# Autodesk Inventor assembly: Outer Wheel
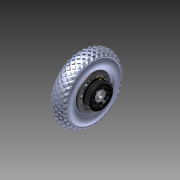
[picture p0: Inventor's stored thumbnail of the model, 180x180]
Saved by Autodesk Inventor 2014 SP1 (Build 180222100, 222)
## iProperties
Created: 2014-01-21
Part Number: Outer Wheel
Document SubType Name: Assembly
Designer: Nick
Author: Nick
## Documents named in this file (4)
- D:\Dropbox\School\PurdueFIRST\PFP Robot\PFP Robot with Cart\Outer Wheel.iam
- D:\Dropbox\School\PurdueFIRST\PFP Robot\PFP Robot with Cart\Pulley.iam
- D:\Dropbox\School\PurdueFIRST\PFP Robot\PFP Robot with Cart\PneumaticWheel_am-0970.iam
- D:\Dropbox\School\PurdueFIRST\PFP Robot\PFP Robot with Cart\6383K234.ipt
## Components (4 placed, 3 different names)
1. Pulley:1 [sub-assembly] — Insert:1, Insert:3, Insert:4
2. PneumaticWheel_am-0970:1 [sub-assembly] — Insert:2, Insert:3, Insert:4
3. 6383K234:1 — Insert:2
4. 6383K234:2 — Insert:1
## Relationships (4: Insert 4)
- Insert:1: Pulley:1 ↔ 6383K234:2
- Insert:2: PneumaticWheel_am-0970:1 ↔ 6383K234:1
- Insert:3 (9.525 mm): Pulley:1 ↔ PneumaticWheel_am-0970:1
- Insert:4 (9.525 mm): Pulley:1 ↔ PneumaticWheel_am-0970:1
